# Autodesk Inventor assembly: payloads
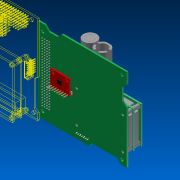
[picture p0: Inventor's stored thumbnail of the model, 180x180]
Saved by Autodesk Inventor 2012 (Build 160160000, 160)
## iProperties
Created: 2015-11-18
Part Number: payloads
Document SubType Name: Assembly
Designer: Alex Becerra
Mass: 90.1266 g
Surface Area: 456.454 cm^2
Volume: 35.4828 cm^3
Density: 2.54001 g/cm^3
Author: Alex Becerra
## Documents named in this file (5)
- C:\Users\Thinkpad\Cubesat SUChAI\Mecanica\Modelo_3D\Placa_payloads\payloads.iam
- C:\Users\Thinkpad\Cubesat SUChAI\Mecanica\Modelo_3D\Placa_payloads\Cam_DespLP\Cam_DespLP.iam
- C:\Users\Thinkpad\Cubesat SUChAI\Mecanica\Modelo_3D\Placa_payloads\Giroscopio\placa_gyro.ipt
- C:\Users\Thinkpad\Cubesat SUChAI\Mecanica\Modelo_3D\Placa_payloads\GPS\GPS.iam
- C:\Users\Thinkpad\Cubesat SUChAI\Mecanica\Modelo_3D\Placa_payloads\Placa_base\Placa_base.iam
## Components (4 placed, 4 different names)
1. Cam_DespLP:1 [sub-assembly] — Mate:7, Flush:1, Flush:2
2. placa_gyro:1 — Mate:4, Mate:5, Mate:6
3. GPS:1 [sub-assembly] — Mate:1, Mate:2, Mate:3
4. Placa_base:1 [sub-assembly] — Mate:1, Mate:2, Mate:3, Mate:4, Mate:5, Mate:6, Mate:7, Flush:1, Flush:2
## Relationships (9: Mate 7, Flush 2)
- Mate:1: GPS:1 ↔ Placa_base:1
- Mate:2: GPS:1 ↔ Placa_base:1
- Mate:3: GPS:1 ↔ Placa_base:1
- Mate:4: placa_gyro:1 ↔ Placa_base:1
- Mate:5: placa_gyro:1 ↔ Placa_base:1
- Mate:6: placa_gyro:1 ↔ Placa_base:1
- Mate:7: Cam_DespLP:1 ↔ Placa_base:1
- Flush:1 (20 mm): Cam_DespLP:1 ↔ Placa_base:1
- Flush:2 (22 mm): Cam_DespLP:1 ↔ Placa_base:1
